# Autodesk Inventor assembly: 2018_chassis
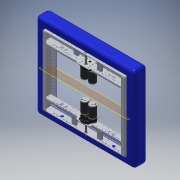
[picture p0: Inventor's stored thumbnail of the model, 180x180]
Saved by Autodesk Inventor 2017 SP1 (Build 210196100, 196)
## iProperties
Created: 2018-01-16
Part Number: 2018_chassis
Description: STEP AP214
Document SubType Name: Assembly
Designer: Ben
Surface Area: 27495 cm^2
Volume: 34872.5 cm^3
Sending System: SolidWorks 2017
Preprocessor: SwSTEP 2.0
Title: 2018_chassis.STEP
Revision Number: ANY
## Documents named in this file (12)
- C:\Users\Ben\Desktop\Projects\2018 Robot\Chassis\2018_chassis.iam
- C:\Users\Ben\Desktop\Projects\2018 Robot\Chassis\am-2951a_AM14U3_Outside_Plate.ipt
- C:\Users\Ben\Desktop\Projects\2018 Robot\Chassis\am-2952a_AM14U3_Inside_Plate.ipt
- C:\Users\Ben\Desktop\Projects\2018 Robot\Chassis\am-3513+AM14U3+End+Plate+27in.ipt
- C:\Users\Ben\Desktop\Projects\2018 Robot\Chassis\TM Housing.ipt
- C:\Users\Ben\Desktop\Projects\2018 Robot\Chassis\R6ZZ Bearing.ipt
- C:\Users\Ben\Desktop\Projects\2018 Robot\Chassis\FR8ZZ Hex Bearing.ipt
- C:\Users\Ben\Desktop\Projects\2018 Robot\Chassis\am-0255+2.5inch+CIM+Motor.ipt
- C:\Users\Ben\Desktop\Projects\2018 Robot\Chassis\am-0801a+Toughbox+Long+Hex+Shaft+With+Magnet.iam
- C:\Users\Ben\Desktop\Projects\2018 Robot\Chassis\inner_rail_support.ipt
- C:\Users\Ben\Desktop\Projects\2018 Robot\Chassis\bumpers.ipt
- C:\Users\Ben\Desktop\Projects\2018 Robot\Chassis\omni wheel.ipt
## Components (29 placed, 26 different names)
1. am-2951a_AM14U3_Outside_Plate_1 — Symmetry:1
2. am-2951a_AM14U3_Outside_Plate_2 — Symmetry:1, Mate:2, Mate:3, Mate:4
3. am-2952a_AM14U3_Inside_Plate_3 — Mate:5, Mate:6, Flush:2, Flush:3
4. am-2952a_AM14U3_Inside_Plate_4 — Flush:4, Flush:5
5. am-3513+AM14U3+End+Plate+27in_5
6. am-3513+AM14U3+End+Plate+27in_6 — Flush:1, Mate:1
7. TM Housing_7
8. TM Housing_8
9. R6ZZ Bearing_9
10. R6ZZ Bearing_10
11. FR8ZZ Hex Bearing_11
12. FR8ZZ Hex Bearing_12
13. FR8ZZ Hex Bearing_13
14. FR8ZZ Hex Bearing_14
15. am-0255+2.5inch+CIM+Motor_15
16. am-0255+2.5inch+CIM+Motor_16
17. am-0801a+Toughbox+Long+Hex+Shaft+With+Magnet_17 [sub-assembly]
18. am-0801a+Toughbox+Long+Hex+Shaft+With+Magnet_18 [sub-assembly]
19. am-0255+2.5inch+CIM+Motor_19
20. am-0255+2.5inch+CIM+Motor_20
21. inner_rail_support_21
22. inner_rail_support_22
23. inner_rail_support_23
24. inner_rail_support_24
25. bumpers:1 — Flush:1, Mate:1, Mate:2
26. omni wheel:1 — Mate:3, Flush:4
27. omni wheel:2 — Mate:4, Flush:5
28. omni wheel:3 — Mate:6, Flush:2
29. omni wheel:4 — Mate:5, Flush:3
## Relationships (12: Mate 6, Flush 5, Symmetry 1)
- Symmetry:1: am-2951a_AM14U3_Outside_Plate_1 ↔ am-2951a_AM14U3_Outside_Plate_2
- Flush:1 (19.05 mm): am-3513+AM14U3+End+Plate+27in_6 ↔ bumpers:1
- Mate:1 (3.175 mm): am-3513+AM14U3+End+Plate+27in_6 ↔ bumpers:1
- Mate:2 (6.35 mm): am-2951a_AM14U3_Outside_Plate_2 ↔ bumpers:1
- Mate:3: am-2951a_AM14U3_Outside_Plate_2 ↔ omni wheel:1
- Mate:4: am-2951a_AM14U3_Outside_Plate_2 ↔ omni wheel:2
- Mate:5: am-2952a_AM14U3_Inside_Plate_3 ↔ omni wheel:4
- Mate:6: am-2952a_AM14U3_Inside_Plate_3 ↔ omni wheel:3
- Flush:2 (38.1 mm): am-2952a_AM14U3_Inside_Plate_3 ↔ omni wheel:3
- Flush:3 (38.1 mm): am-2952a_AM14U3_Inside_Plate_3 ↔ omni wheel:4
- Flush:4 (38.1 mm): am-2952a_AM14U3_Inside_Plate_4 ↔ omni wheel:1
- Flush:5 (38.1 mm): am-2952a_AM14U3_Inside_Plate_4 ↔ omni wheel:2
